# Autodesk Inventor assembly: SegaStraightAssembly01
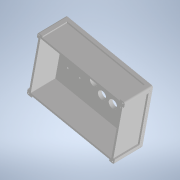
[picture p0: Inventor's stored thumbnail of the model, 180x180]
Saved by Autodesk Inventor 2022 (Build 260153000, 153)
## iProperties
Created: 2023-03-05
Part Number: SegaStraightAssembly01
Document SubType Name: Assembly
Designer: Bunny
Author: Bunny
## Documents named in this file (7)
- C:\Users\Bunny\OneDrive - The University of Melbourne\project\controller\model\SegaStraightAssembly01.iam
- C:\Users\Bunny\OneDrive - The University of Melbourne\project\controller\model\sega_straight.ipt
- C:\Users\Bunny\OneDrive - The University of Melbourne\project\controller\model\cab_L_F.ipt
- C:\Users\Bunny\OneDrive - The University of Melbourne\project\controller\model\cab_L_B.ipt
- C:\Users\Bunny\OneDrive - The University of Melbourne\project\controller\model\cab_L_L.ipt
- C:\Users\Bunny\OneDrive - The University of Melbourne\project\controller\model\Corner.ipt
- C:\Users\Bunny\OneDrive - The University of Melbourne\project\controller\model\sega_straight_b1.ipt
## Components (10 placed, 6 different names)
1. sega_straight:1 — Mate:27, Mate:28, Mate:29
2. cab_L_F:1 — Mate:1, Mate:3, Mate:15, Mate:16, Mate:24
3. cab_L_B:1 — Mate:8, Mate:9, Mate:10, Mate:12, Mate:13, Mate:14, Mate:23
4. cab_L_L:1 — Mate:2, Mate:4, Mate:5, Mate:6, Mate:7, Mate:11
5. cab_L_L:2 — Mate:17, Mate:18, Mate:19
6. Corner:1 — Mate:1, Mate:2, Mate:3, Mate:4, Mate:26
7. Corner:2 — Mate:5, Mate:6, Mate:7, Mate:8, Mate:9, Mate:10, Mate:11, Mate:23
8. Corner:3 — Mate:12, Mate:13, Mate:14, Mate:19
9. Corner:4 — Mate:15, Mate:16, Mate:17, Mate:18, Mate:25
10. sega_straight_b1:1 — Mate:24, Mate:25, Mate:26, Mate:27, Mate:28, Mate:29
## Relationships (26: Mate 26)
- Mate:1: cab_L_F:1 ↔ Corner:1
- Mate:2: cab_L_L:1 ↔ Corner:1
- Mate:3: cab_L_F:1 ↔ Corner:1
- Mate:4: cab_L_L:1 ↔ Corner:1
- Mate:5: cab_L_L:1 ↔ Corner:2
- Mate:6: cab_L_L:1 ↔ Corner:2
- Mate:7: cab_L_L:1 ↔ Corner:2
- Mate:8: cab_L_B:1 ↔ Corner:2
- Mate:9: cab_L_B:1 ↔ Corner:2
- Mate:10: cab_L_B:1 ↔ Corner:2
- Mate:11: cab_L_L:1 ↔ Corner:2
- Mate:12: cab_L_B:1 ↔ Corner:3
- Mate:13: cab_L_B:1 ↔ Corner:3
- Mate:14: cab_L_B:1 ↔ Corner:3
- Mate:15: cab_L_F:1 ↔ Corner:4
- Mate:16: cab_L_F:1 ↔ Corner:4
- Mate:17: cab_L_L:2 ↔ Corner:4
- Mate:18: cab_L_L:2 ↔ Corner:4
- Mate:19: cab_L_L:2 ↔ Corner:3
- Mate:23: cab_L_B:1 ↔ Corner:2
- Mate:24: cab_L_F:1 ↔ sega_straight_b1:1
- Mate:25: Corner:4 ↔ sega_straight_b1:1
- Mate:26: Corner:1 ↔ sega_straight_b1:1
- Mate:27: sega_straight:1 ↔ sega_straight_b1:1
- Mate:28: sega_straight:1 ↔ sega_straight_b1:1
- Mate:29: sega_straight:1 ↔ sega_straight_b1:1
## Named parameters: BoxLength = 250 mm, BoxHeight = 80 mm, BoxWidth = 200 mm, SheetThickness = 6 mm, CornerOffset = 5 mm
